# Autodesk Inventor assembly: Engine Assembly
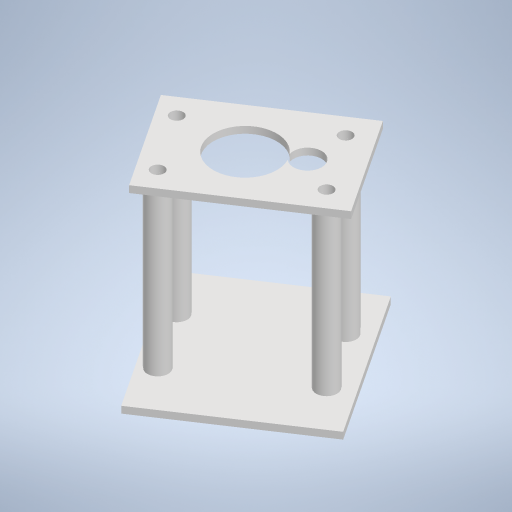
[picture p0: Inventor's stored thumbnail of the model, 512x512]
Saved by Autodesk Inventor 2023 (Build 270158000, 158)
## iProperties
Created: 2023-02-13
Part Number: Engine Assembly
Document SubType Name: Assembly
Designer: tommy
Author: tommy
## Documents named in this file (4)
- C:\Users\tommy\Documents\Repositories\Steam-Engine\Les Proper Steam Engine\CAD\Engine Assembly.iam
- C:\Users\tommy\Documents\Repositories\Steam-Engine\Les Proper Steam Engine\CAD\Base Bottom.ipt
- C:\Users\tommy\Documents\Repositories\Steam-Engine\Les Proper Steam Engine\CAD\Base Top.ipt
- C:\Users\tommy\Documents\Repositories\Steam-Engine\Les Proper Steam Engine\CAD\Frame Post.ipt
## Components (6 placed, 3 different names)
1. Base Bottom:1 — Mate:9, Mate:10, Mate:11
2. Base Top:1 — Mate:1, Mate:2, Mate:3, Mate:4, Mate:5, Mate:6, Mate:7, Mate:8
3. Frame Post:1 — Mate:1, Mate:2
4. Frame Post:2 — Mate:4, Mate:6, Mate:9, Mate:10
5. Frame Post:3 — Mate:3, Mate:7, Mate:11
6. Frame Post:4 — Mate:5, Mate:8
## Relationships (11: Mate 11)
- Mate:1: Base Top:1 ↔ Frame Post:1
- Mate:2: Base Top:1 ↔ Frame Post:1
- Mate:3: Base Top:1 ↔ Frame Post:3
- Mate:4: Base Top:1 ↔ Frame Post:2
- Mate:5: Base Top:1 ↔ Frame Post:4
- Mate:6: Base Top:1 ↔ Frame Post:2
- Mate:7: Base Top:1 ↔ Frame Post:3
- Mate:8: Base Top:1 ↔ Frame Post:4
- Mate:9: Base Bottom:1 ↔ Frame Post:2
- Mate:10: Base Bottom:1 ↔ Frame Post:2
- Mate:11: Base Bottom:1 ↔ Frame Post:3
